# Autodesk Inventor assembly: 4_6_Gear_Assembly
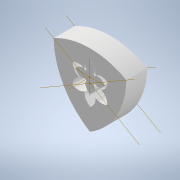
[picture p0: Inventor's stored thumbnail of the model, 180x180]
Saved by Autodesk Inventor 2021 (Build 250183000, 183)
## iProperties
Created: 2021-03-25
Part Number: 4_6_Gear_Assembly
Document SubType Name: Assembly
Designer: lucia
Author: lucia
## Documents named in this file (3)
- E:\Documents\Inventor\Fixed Rotor Wankel Engine\Parts\4_6_Gear_Assembly.iam
- E:\Documents\Inventor\Fixed Rotor Wankel Engine\Parts\Rotor_Geared_6t.ipt
- E:\Documents\Inventor\Fixed Rotor Wankel Engine\Parts\Gear_4t.ipt
## Components (2 placed, 2 different names)
1. Rotor_Geared_6t:1 — Flush:1, Flush:2, Mate:1, Mate:2, Mate:3, Mate:4, Mate:5, Mate:6, Mate:7, Mate:8, Rotation:1
2. Gear_4t:1 — Flush:2, Mate:16, Mate:17, Mate:18, Mate:19, Mate:20, Mate:21, Mate:22, Mate:23, Rotation:1
## Relationships (34: Mate 31, Flush 2, RelateRotation 1)
- Flush:1: Rotor_Geared_6t:1
- Flush:2: Rotor_Geared_6t:1 ↔ Gear_4t:1
- Mate:1: Rotor_Geared_6t:1
- Mate:2: Rotor_Geared_6t:1
- Mate:3: Rotor_Geared_6t:1
- Mate:4: Rotor_Geared_6t:1
- Mate:5: Rotor_Geared_6t:1
- Mate:6: Rotor_Geared_6t:1
- Mate:7: Rotor_Geared_6t:1
- Mate:8: Rotor_Geared_6t:1
- Mate:9
- Mate:10
- Mate:11
- Mate:12
- Mate:13
- Mate:14
- Mate:15
- Mate:16: Gear_4t:1
- Mate:17: Gear_4t:1
- Mate:18: Gear_4t:1
- Mate:19: Gear_4t:1
- Mate:20: Gear_4t:1
- Mate:21: Gear_4t:1
- Mate:22: Gear_4t:1
- Mate:23: Gear_4t:1
- Mate:24
- Mate:25
- Mate:26
- Mate:27
- Mate:28
- Mate:29
- Mate:30
- Mate:31 (13.208 mm)
- Rotation:1 [RelateRotation] (0.6667 ul): Rotor_Geared_6t:1 ↔ Gear_4t:1
